# Autodesk Inventor assembly: joint4
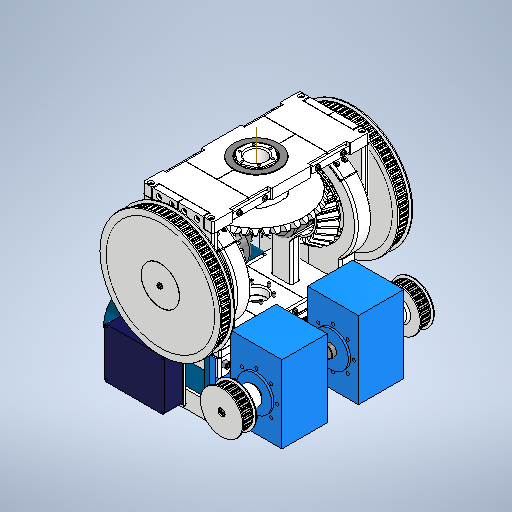
[picture p0: Inventor's stored thumbnail of the model, 512x512]
Saved by Autodesk Inventor 2025.3 (Build 293356030, 356C)
## iProperties
Created: 2025-08-31
Part Number: joint4
Document SubType Name: Assembly
Designer: MSI
Mass: 17943.2 g
Surface Area: 11658.9 cm^2
Volume: 6898.44 cm^3
Density: 2.60106 g/cm^3
Author: MSI
## Documents named in this file (23)
- C:\Users\MSI\Desktop\Project\3. 로봇팔\Robot Arm Model\joint3\joint3.iam
- C:\Users\MSI\Desktop\Project\3. 로봇팔\Robot Arm Model\Robot_Arm_6_v1\encoder.ipt
- C:\Users\MSI\Desktop\Project\3. 로봇팔\Robot Arm Model\joint3\joint3_meteor.iam
- C:\Users\MSI\Desktop\Project\3. 로봇팔\Robot Arm Model\joint3\motor.iam
- C:\Users\MSI\Desktop\Project\3. 로봇팔\Robot Arm Model\Robot_Arm_6_v1\C-E6810ZZ_Autodesk_Inventor_2024_20250921\C-E6810ZZ.ipt
- C:\Users\MSI\Desktop\Project\3. 로봇팔\Robot Arm Model\Robot_Arm_6_v1\NTN_GS81110OuterRings\GS81110Outer Rings.ipt
- C:\Users\MSI\Desktop\Project\3. 로봇팔\Robot Arm Model\Robot_Arm_6_v1\belt_axis.ipt
- C:\Users\MSI\Desktop\Project\3. 로봇팔\Robot Arm Model\Robot_Arm_6_v1\joint3\디자인 액셀러레이터\베벨 기어1.iam
- C:\Users\MSI\Desktop\Project\3. 로봇팔\Robot Arm Model\Robot_Arm_6_v1\joint3\디자인 액셀러레이터\베벨 기어11.ipt
- C:\Users\MSI\Desktop\Project\3. 로봇팔\Robot Arm Model\joint3\encoder_supporter.ipt
- C:\Users\MSI\Desktop\Project\3. 로봇팔\Robot Arm Model\joint3\joint3_washer2.ipt
- C:\Users\MSI\Desktop\Project\3. 로봇팔\Robot Arm Model\joint3\joint3_washer1.ipt
- C:\Users\MSI\Desktop\Project\3. 로봇팔\Robot Arm Model\joint3\C-E6806ZZ_Autodesk_Inventor_2024_20251124\C-E6806ZZ.ipt
- C:\Users\MSI\Desktop\Project\3. 로봇팔\Robot Arm Model\joint3\joint3_axis3_washer.ipt
- C:\Users\MSI\Desktop\Project\3. 로봇팔\Robot Arm Model\joint3\joint3_asix4.ipt
- C:\Users\MSI\Documents\Inventor\Content Center Files\R2025\ko-KR\KS B 1023  H (2)\KS B 1023 - A  M 4 x 16 - H(1).ipt
- C:\Users\MSI\Desktop\Project\3. 로봇팔\Robot Arm Model\joint3\HTPA72S8M150-A-H20_Inventor\HTPA72S8M150-A-H20.iam
- C:\Users\MSI\Desktop\Project\3. 로봇팔\Robot Arm Model\joint3\BLPA24S8M150-A-H12_Autodesk_Inventor_2024_20251124\AIS2024\BLPA24S8M150-A-H12_b.ipt
- C:\Users\MSI\Desktop\Project\3. 로봇팔\Robot Arm Model\joint3\joint3_base.iam
- C:\Users\MSI\Desktop\Project\3. 로봇팔\Robot Arm Model\joint3\joint3_frame.iam
- C:\Users\MSI\Documents\Inventor\Content Center Files\R2025\ko-KR\KS B 1023  H (2)\KS B 1023 - A  M 4 x 30 - H(1).ipt
- C:\Users\MSI\Documents\Inventor\Content Center Files\R2025\ko-KR\KS B 1023  H (2)\KS B 1023 - A  M 6 x 16 - H(1).ipt
- C:\Users\MSI\Documents\Inventor\Content Center Files\R2025\ko-KR\KS B 1023  H (2)\KS B 1023 - A  M 4 x 25 - H(1).ipt
## Components (67 placed, 22 different names)
1. motor:1 [sub-assembly] — 메이트:7, 메이트:8, 메이트:9, 각도:3, 메이트:15, 메이트:16, 삽입:36, 각도:24, 각도:25, 삽입:37, 삽입:46, 삽입:48
2. joint3_base:1 [sub-assembly] — 메이트:7, 메이트:1, 메이트:2, 메이트:3, 삽입:11, 삽입:12, 삽입:29, 삽입:30, 메이트:15, 메이트:16, 메이트:18, 메이트:20, 메이트:21, 메이트:23, 메이트:24, 삽입:44, 삽입:45
3. joint3_frame:1 [sub-assembly] — 메이트:5, 메이트:6, 삽입:18, 삽입:19, 삽입:22, 삽입:23, 삽입:26, 삽입:15, 삽입:33
4. encoder:1 — 삽입:10, 메이트:10
5. encoder:2 — 삽입:28, 메이트:14
6. belt_axis:1 — 삽입:17, 메이트:11, 각도:19, 각도:20, 삽입:32, 각도:21
7. belt_axis:2 — 삽입:31, 메이트:17, 각도:22, 삽입:35, 각도:23
8. joint3_meteor:1 [sub-assembly] — 삽입:13, 삽입:17, 메이트:11, 메이트:22, 메이트:23, 메이트:24, 삽입:38
9. joint3_meteor:2 [sub-assembly] — 삽입:14, 삽입:31, 메이트:17, 메이트:18, 메이트:19, 메이트:20, 메이트:21, 삽입:39
10. GS81110Outer Rings:1 — 삽입:23
11. C-E6810ZZ:1 — 삽입:24, 삽입:25
12. GS81110Outer Rings:2 — 삽입:26
13. 베벨 기어:1 [sub-assembly] — 메이트:1, 메이트:2, 메이트:4, 메이트:5, 삽입:27, 메이트:13, 메이트:10, 메이트:22, 삽입:47
14. 베벨 기어1:5 — 메이트:3, 메이트:4, 메이트:6, 메이트:19
15. encoder_supporter:1 — 삽입:28, 메이트:14, 삽입:29, 삽입:30
16. encoder_supporter:2 — 삽입:10, 삽입:11, 삽입:12
17. joint3_washer2:1 — 삽입:13, 각도:19
18. joint3_washer2:2 — 삽입:14, 각도:22
19. joint3_washer1:1 — 삽입:15, 각도:20
20. C-E6806ZZ:1 — 삽입:18
21. C-E6806ZZ:2 — 삽입:19
22. joint3_axis3_washer:1 — 삽입:22, 삽입:24
23. joint3_axis3_washer:2 — 삽입:25
24. joint3_asix4:1 — 삽입:27, 메이트:13
25. HTPA72S8M150-A-H20:1 [sub-assembly] — 삽입:32, 각도:21, 삽입:41
26. KS B 1023 H - 미터 A  M 4 x 16 - H:2 — 삽입:41
27. joint3_washer1:2 — 삽입:33
28. HTPA72S8M150-A-H20:2 [sub-assembly] — 삽입:35, 각도:23, 삽입:40
29. KS B 1023 H - 미터 A  M 4 x 16 - H:1 — 삽입:40
30. BLPA24S8M150-A-H12_b:1 — 삽입:36, 각도:24, 삽입:42
31. BLPA24S8M150-A-H12_b:2 — 각도:25, 삽입:37, 삽입:43
32. KS B 1023 H - 미터 A  M 6 x 16 - H:1 — 삽입:42
33. KS B 1023 H - 미터 A  M 6 x 16 - H:2 — 삽입:43
34. KS B 1023 H - 미터 A  M 4 x 30 - H:2 — 삽입:39
35. KS B 1023 H - 미터 A  M 4 x 30 - H:1 — 삽입:38
36. KS B 1023 H - 미터 A  M 4 x 30 - H:3
37. KS B 1023 H - 미터 A  M 4 x 30 - H:4
38. KS B 1023 H - 미터 A  M 4 x 30 - H:5
39. KS B 1023 H - 미터 A  M 4 x 30 - H:6
40. KS B 1023 H - 미터 A  M 4 x 30 - H:7
41. KS B 1023 H - 미터 A  M 4 x 30 - H:8
42. KS B 1023 H - 미터 A  M 4 x 16 - H:3 — 삽입:44
43. KS B 1023 H - 미터 A  M 4 x 16 - H:4 — 삽입:45
44. KS B 1023 H - 미터 A  M 4 x 16 - H:5
45. KS B 1023 H - 미터 A  M 4 x 16 - H:6
46. KS B 1023 H - 미터 A  M 4 x 16 - H:7
47. KS B 1023 H - 미터 A  M 4 x 16 - H:8
48. KS B 1023 H - 미터 A  M 4 x 16 - H:9
49. KS B 1023 H - 미터 A  M 4 x 16 - H:10
50. KS B 1023 H - 미터 A  M 4 x 25 - H:1 — 삽입:46
51. KS B 1023 H - 미터 A  M 4 x 25 - H:3 — 삽입:48
52. KS B 1023 H - 미터 A  M 4 x 25 - H:2 — 삽입:47
53. KS B 1023 H - 미터 A  M 4 x 25 - H:4
54. KS B 1023 H - 미터 A  M 4 x 25 - H:5
55. KS B 1023 H - 미터 A  M 4 x 25 - H:6
56. KS B 1023 H - 미터 A  M 4 x 25 - H:7
57. KS B 1023 H - 미터 A  M 4 x 25 - H:8
58. KS B 1023 H - 미터 A  M 4 x 25 - H:9
59. KS B 1023 H - 미터 A  M 4 x 25 - H:10
60. KS B 1023 H - 미터 A  M 4 x 25 - H:11
61. KS B 1023 H - 미터 A  M 4 x 25 - H:12
62. KS B 1023 H - 미터 A  M 4 x 25 - H:13
63. KS B 1023 H - 미터 A  M 4 x 25 - H:14
64. KS B 1023 H - 미터 A  M 4 x 25 - H:15
65. KS B 1023 H - 미터 A  M 4 x 25 - H:16
66. KS B 1023 H - 미터 A  M 4 x 25 - H:17
67. KS B 1023 H - 미터 A  M 4 x 25 - H:18
## Component patterns: (4 elements, first: KS B 1023 H - 미터 A  M 4 x 30 - H:2 + KS B 1023 H - 미터 A  M 4 x 30 - H:1), (4 elements, first: KS B 1023 H - 미터 A  M 4 x 16 - H:3 + KS B 1023 H - 미터 A  M 4 x 16 - H:4), (6 elements, first: KS B 1023 H - 미터 A  M 4 x 25 - H:1 + KS B 1023 H - 미터 A  M 4 x 25 - H:3 + KS B 1023 H - 미터 A  M 4 x 25 - H:2)
## Relationships (66: Insert 35, Mate 23, Angle 8)
- 메이트:7 [Mate]: motor:1 ↔ joint3_base:1
- 메이트:1 [Mate]: joint3_base:1 ↔ 베벨 기어:1
- 메이트:2 [Mate]: joint3_base:1 ↔ 베벨 기어:1
- 메이트:3 [Mate]: joint3_base:1 ↔ 베벨 기어1:5
- 메이트:4 [Mate]: 베벨 기어:1 ↔ 베벨 기어1:5
- 메이트:5 [Mate]: joint3_frame:1 ↔ 베벨 기어:1
- 메이트:6 [Mate]: joint3_frame:1 ↔ 베벨 기어1:5
- 메이트:8 [Mate]: motor:1
- 메이트:9 [Mate]: motor:1
- 각도:3 [Angle] (0 deg): motor:1
- 삽입:10 [Insert]: encoder:1 ↔ encoder_supporter:2
- 삽입:11 [Insert]: joint3_base:1 ↔ encoder_supporter:2
- 메이트:10 [Mate]: encoder:1 ↔ 베벨 기어:1
- 삽입:12 [Insert]: joint3_base:1 ↔ encoder_supporter:2
- 삽입:13 [Insert]: joint3_meteor:1 ↔ joint3_washer2:1
- 삽입:14 [Insert]: joint3_meteor:2 ↔ joint3_washer2:2
- 삽입:15 [Insert] (-1.25 mm): joint3_frame:1 ↔ joint3_washer1:1
- 삽입:17 [Insert]: belt_axis:1 ↔ joint3_meteor:1
- 메이트:11 [Mate]: belt_axis:1 ↔ joint3_meteor:1
- 삽입:18 [Insert]: joint3_frame:1 ↔ C-E6806ZZ:1
- 삽입:19 [Insert]: joint3_frame:1 ↔ C-E6806ZZ:2
- 삽입:22 [Insert]: joint3_frame:1 ↔ joint3_axis3_washer:1
- 삽입:23 [Insert]: joint3_frame:1 ↔ GS81110Outer Rings:1
- 삽입:24 [Insert]: C-E6810ZZ:1 ↔ joint3_axis3_washer:1
- 삽입:25 [Insert]: C-E6810ZZ:1 ↔ joint3_axis3_washer:2
- 삽입:26 [Insert]: joint3_frame:1 ↔ GS81110Outer Rings:2
- 삽입:27 [Insert]: 베벨 기어:1 ↔ joint3_asix4:1
- 메이트:13 [Mate]: 베벨 기어:1 ↔ joint3_asix4:1
- 삽입:28 [Insert]: encoder:2 ↔ encoder_supporter:1
- 메이트:14 [Mate]: encoder:2 ↔ encoder_supporter:1
- 삽입:29 [Insert]: joint3_base:1 ↔ encoder_supporter:1
- 삽입:30 [Insert]: joint3_base:1 ↔ encoder_supporter:1
- 메이트:15 [Mate]: motor:1 ↔ joint3_base:1
- 메이트:16 [Mate]: motor:1 ↔ joint3_base:1
- 삽입:31 [Insert]: belt_axis:2 ↔ joint3_meteor:2
- 메이트:17 [Mate]: belt_axis:2 ↔ joint3_meteor:2
- 각도:19 [Angle] (0 deg): belt_axis:1 ↔ joint3_washer2:1
- 각도:20 [Angle] (0 deg): belt_axis:1 ↔ joint3_washer1:1
- 삽입:32 [Insert]: belt_axis:1 ↔ HTPA72S8M150-A-H20:1
- 각도:21 [Angle] (0 deg): belt_axis:1 ↔ HTPA72S8M150-A-H20:1
- 각도:22 [Angle] (0 deg): belt_axis:2 ↔ joint3_washer2:2
- 삽입:33 [Insert] (-1.25 mm): joint3_frame:1 ↔ joint3_washer1:2
- 삽입:35 [Insert]: belt_axis:2 ↔ HTPA72S8M150-A-H20:2
- 각도:23 [Angle] (0 deg): belt_axis:2 ↔ HTPA72S8M150-A-H20:2
- 삽입:36 [Insert]: motor:1 ↔ BLPA24S8M150-A-H12_b:1
- 각도:24 [Angle] (180 deg): motor:1 ↔ BLPA24S8M150-A-H12_b:1
- 각도:25 [Angle] (0 deg): motor:1 ↔ BLPA24S8M150-A-H12_b:2
- 삽입:37 [Insert]: motor:1 ↔ BLPA24S8M150-A-H12_b:2
- 메이트:18 [Mate]: joint3_base:1 ↔ joint3_meteor:2
- 메이트:19 [Mate]: joint3_meteor:2 ↔ 베벨 기어1:5
- 메이트:20 [Mate]: joint3_base:1 ↔ joint3_meteor:2
- 메이트:21 [Mate]: joint3_base:1 ↔ joint3_meteor:2
- 메이트:22 [Mate]: joint3_meteor:1 ↔ 베벨 기어:1
- 메이트:23 [Mate]: joint3_base:1 ↔ joint3_meteor:1
- 메이트:24 [Mate]: joint3_base:1 ↔ joint3_meteor:1
- 삽입:38 [Insert]: joint3_meteor:1 ↔ KS B 1023 H - 미터 A  M 4 x 30 - H:1
- 삽입:39 [Insert]: joint3_meteor:2 ↔ KS B 1023 H - 미터 A  M 4 x 30 - H:2
- 삽입:40 [Insert]: HTPA72S8M150-A-H20:2 ↔ KS B 1023 H - 미터 A  M 4 x 16 - H:1
- 삽입:41 [Insert]: HTPA72S8M150-A-H20:1 ↔ KS B 1023 H - 미터 A  M 4 x 16 - H:2
- 삽입:42 [Insert]: BLPA24S8M150-A-H12_b:1 ↔ KS B 1023 H - 미터 A  M 6 x 16 - H:1
- 삽입:43 [Insert]: BLPA24S8M150-A-H12_b:2 ↔ KS B 1023 H - 미터 A  M 6 x 16 - H:2
- 삽입:44 [Insert]: joint3_base:1 ↔ KS B 1023 H - 미터 A  M 4 x 16 - H:3
- 삽입:45 [Insert]: joint3_base:1 ↔ KS B 1023 H - 미터 A  M 4 x 16 - H:4
- 삽입:46 [Insert]: motor:1 ↔ KS B 1023 H - 미터 A  M 4 x 25 - H:1
- 삽입:47 [Insert]: 베벨 기어:1 ↔ KS B 1023 H - 미터 A  M 4 x 25 - H:2
- 삽입:48 [Insert]: motor:1 ↔ KS B 1023 H - 미터 A  M 4 x 25 - H:3
## Named parameters: d145_d112 = -1.25 mm
